# Autodesk Inventor assembly: 膝_1
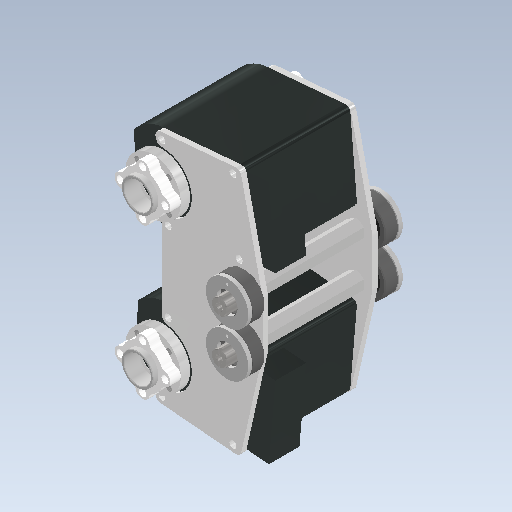
[picture p0: Inventor's stored thumbnail of the model, 512x512]
Saved by Autodesk Inventor 2020 (Build 240168000, 168)
## iProperties
Created: 2021-09-06
Part Number: 膝_1
Document SubType Name: Assembly
Designer: Masato
Author: Masato
## Documents named in this file (11)
- C:\Users\Masato\Desktop\最新版\OpenPlatform_ver3_0\下半身\膝\膝_1.iam
- C:\Users\Masato\Desktop\最新版\OpenPlatform_ver3_0\下半身\膝\膝_メインフレーム_1.ipt
- C:\Users\Masato\Desktop\最新版\OpenPlatform_ver3_0\Ready_Made\B3M11xx.ipt
- C:\Users\Masato\Desktop\最新版\OpenPlatform_ver3_0\下半身\リンク\リンク_ふくらはぎ_サブフレーム_1_4.ipt
- C:\Users\Masato\Desktop\最新版\OpenPlatform_ver3_0\Ready_Made\free_horn.ipt
- C:\Users\Masato\Desktop\最新版\OpenPlatform_ver3_0\Ready_Made\WSSS12-10-6.ipt
- C:\Users\Masato\Desktop\最新版\OpenPlatform_ver3_0\Ready_Made\SLSBF6-39_5-M3-N3.ipt
- C:\Users\Masato\Desktop\最新版\OpenPlatform_ver3_0\Ready_Made\BRU-309_5S.ipt
- C:\Users\Masato\Desktop\最新版\OpenPlatform_ver3_0\Ready_Made\UUW-0312-10BH.ipt
- C:\Users\Masato\Desktop\最新版\OpenPlatform_ver3_0\Ready_Made\GSB-081605.ipt
- C:\Users\Masato\Desktop\最新版\OpenPlatform_ver3_0\Ready_Made\LFW-0815.ipt
## Components (32 placed, 10 different names)
1. 膝_メインフレーム_1:1 — 挿入:1, 挿入:2, 挿入:3, 挿入:4, 挿入:5, 挿入:6, 挿入:7, 挿入:8, メイト:1, 挿入:41, 挿入:42, 挿入:45, 挿入:46
2. 膝_メインフレーム_1:2 — 挿入:9, 挿入:10, 挿入:11, 挿入:12, 挿入:13, 挿入:14, 挿入:15, 挿入:16, 挿入:43, 挿入:44, 挿入:47, 挿入:48
3. B3M11xx:1 — 挿入:1, 挿入:2, 挿入:5, 挿入:6, 挿入:9, 挿入:10, 挿入:15, 挿入:16, 挿入:31, 挿入:33
4. B3M11xx:2 — 挿入:3, 挿入:4, 挿入:7, 挿入:8, 挿入:11, 挿入:12, 挿入:13, 挿入:14, 挿入:32, 挿入:34
5. リンク_ふくらはぎ_サブフレーム_1_4:1 — 挿入:32, 挿入:38
6. リンク_ふくらはぎ_サブフレーム_1_4:2 — 挿入:31, 挿入:37
7. リンク_ふくらはぎ_サブフレーム_1_4:3 — 挿入:36, 挿入:39
8. リンク_ふくらはぎ_サブフレーム_1_4:4 — 挿入:35, 挿入:40
9. free_horn:1 — 挿入:33, 挿入:35
10. free_horn:2 — 挿入:34, 挿入:36
11. WSSS12-10-6:1 — 挿入:37
12. WSSS12-10-6:2 — 挿入:38
13. WSSS12-10-6:3 — 挿入:39
14. WSSS12-10-6:4 — 挿入:40
15. SLSBF6-39_5-M3-N3:1 — 挿入:41, 挿入:43
16. SLSBF6-39_5-M3-N3:2 — 挿入:42, 挿入:44
17. BRU-309_5S:1 — 挿入:49
18. BRU-309_5S:2 — 挿入:52
19. BRU-309_5S:3 — 挿入:51
20. BRU-309_5S:4 — 挿入:50
21. UUW-0312-10BH:1 — 挿入:45, 挿入:51, 挿入:53
22. UUW-0312-10BH:2 — 挿入:46, 挿入:52, 挿入:54
23. UUW-0312-10BH:3 — 挿入:47, 挿入:49, 挿入:55
24. UUW-0312-10BH:4 — 挿入:48, 挿入:50, 挿入:56
25. GSB-081605:1 — 挿入:54, 挿入:58
26. GSB-081605:2 — 挿入:56, 挿入:60
27. GSB-081605:3 — 挿入:55, 挿入:59
28. GSB-081605:4 — 挿入:53, 挿入:57
29. LFW-0815:1 — 挿入:57
30. LFW-0815:2 — 挿入:58
31. LFW-0815:3 — 挿入:59
32. LFW-0815:4 — 挿入:60
## Relationships (47: Insert 46, Mate 1)
- 挿入:1 [Insert]: 膝_メインフレーム_1:1 ↔ B3M11xx:1
- 挿入:2 [Insert]: 膝_メインフレーム_1:1 ↔ B3M11xx:1
- 挿入:3 [Insert]: 膝_メインフレーム_1:1 ↔ B3M11xx:2
- 挿入:4 [Insert]: 膝_メインフレーム_1:1 ↔ B3M11xx:2
- 挿入:5 [Insert]: 膝_メインフレーム_1:1 ↔ B3M11xx:1
- 挿入:6 [Insert]: 膝_メインフレーム_1:1 ↔ B3M11xx:1
- 挿入:7 [Insert]: 膝_メインフレーム_1:1 ↔ B3M11xx:2
- 挿入:8 [Insert]: 膝_メインフレーム_1:1 ↔ B3M11xx:2
- 挿入:9 [Insert]: 膝_メインフレーム_1:2 ↔ B3M11xx:1
- 挿入:10 [Insert]: 膝_メインフレーム_1:2 ↔ B3M11xx:1
- 挿入:11 [Insert]: 膝_メインフレーム_1:2 ↔ B3M11xx:2
- 挿入:12 [Insert]: 膝_メインフレーム_1:2 ↔ B3M11xx:2
- 挿入:13 [Insert]: 膝_メインフレーム_1:2 ↔ B3M11xx:2
- 挿入:14 [Insert]: 膝_メインフレーム_1:2 ↔ B3M11xx:2
- 挿入:15 [Insert]: 膝_メインフレーム_1:2 ↔ B3M11xx:1
- 挿入:16 [Insert]: 膝_メインフレーム_1:2 ↔ B3M11xx:1
- 挿入:31 [Insert]: B3M11xx:1 ↔ リンク_ふくらはぎ_サブフレーム_1_4:2
- 挿入:32 [Insert]: B3M11xx:2 ↔ リンク_ふくらはぎ_サブフレーム_1_4:1
- 挿入:33 [Insert]: B3M11xx:1 ↔ free_horn:1
- 挿入:34 [Insert]: B3M11xx:2 ↔ free_horn:2
- 挿入:35 [Insert]: リンク_ふくらはぎ_サブフレーム_1_4:4 ↔ free_horn:1
- 挿入:36 [Insert]: リンク_ふくらはぎ_サブフレーム_1_4:3 ↔ free_horn:2
- 挿入:37 [Insert]: リンク_ふくらはぎ_サブフレーム_1_4:2 ↔ WSSS12-10-6:1
- 挿入:38 [Insert]: リンク_ふくらはぎ_サブフレーム_1_4:1 ↔ WSSS12-10-6:2
- 挿入:39 [Insert]: リンク_ふくらはぎ_サブフレーム_1_4:3 ↔ WSSS12-10-6:3
- 挿入:40 [Insert]: リンク_ふくらはぎ_サブフレーム_1_4:4 ↔ WSSS12-10-6:4
- メイト:1 [Mate] (19.75 mm): 膝_メインフレーム_1:1
- 挿入:41 [Insert]: 膝_メインフレーム_1:1 ↔ SLSBF6-39_5-M3-N3:1
- 挿入:42 [Insert]: 膝_メインフレーム_1:1 ↔ SLSBF6-39_5-M3-N3:2
- 挿入:43 [Insert]: 膝_メインフレーム_1:2 ↔ SLSBF6-39_5-M3-N3:1
- 挿入:44 [Insert]: 膝_メインフレーム_1:2 ↔ SLSBF6-39_5-M3-N3:2
- 挿入:45 [Insert]: 膝_メインフレーム_1:1 ↔ UUW-0312-10BH:1
- 挿入:46 [Insert]: 膝_メインフレーム_1:1 ↔ UUW-0312-10BH:2
- 挿入:47 [Insert]: 膝_メインフレーム_1:2 ↔ UUW-0312-10BH:3
- 挿入:48 [Insert]: 膝_メインフレーム_1:2 ↔ UUW-0312-10BH:4
- 挿入:49 [Insert]: BRU-309_5S:1 ↔ UUW-0312-10BH:3
- 挿入:50 [Insert]: BRU-309_5S:4 ↔ UUW-0312-10BH:4
- 挿入:51 [Insert]: BRU-309_5S:3 ↔ UUW-0312-10BH:1
- 挿入:52 [Insert]: BRU-309_5S:2 ↔ UUW-0312-10BH:2
- 挿入:53 [Insert]: UUW-0312-10BH:1 ↔ GSB-081605:4
- 挿入:54 [Insert]: UUW-0312-10BH:2 ↔ GSB-081605:1
- 挿入:55 [Insert]: UUW-0312-10BH:3 ↔ GSB-081605:3
- 挿入:56 [Insert]: UUW-0312-10BH:4 ↔ GSB-081605:2
- 挿入:57 [Insert]: GSB-081605:4 ↔ LFW-0815:1
- 挿入:58 [Insert]: GSB-081605:1 ↔ LFW-0815:2
- 挿入:59 [Insert]: GSB-081605:3 ↔ LFW-0815:3
- 挿入:60 [Insert]: GSB-081605:2 ↔ LFW-0815:4
